# Autodesk Inventor assembly: ASY ДМФ лоток 050 илоотвод v2.0
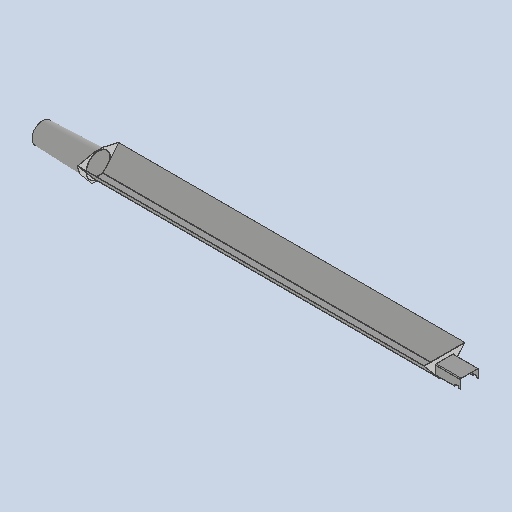
[picture p0: Inventor's stored thumbnail of the model, 512x512]
Saved by Autodesk Inventor 2026.2 (Build 302298000, 298)
## iProperties
Created: 2024-05-14
Part Number: ASY ДМФ лоток 050 илоотвод v2.0
Document SubType Name: Assembly
Designer: admin
Author: admin
## Documents named in this file (6)
- C:\Users\admin\Documents\Inventor\DMF-Disk-Micro-Filter\ASY ДМФ лоток 050 илоотвод v2.0.iam
- C:\Users\admin\Documents\Inventor\DMF-Disk-Micro-Filter\ДМФ 051 лоток илоотвод v2.0.ipt
- C:\Users\admin\Documents\Inventor\DMF-Disk-Micro-Filter\ДМФ 052 торец лотка кормовой v2.0.ipt
- C:\Users\admin\Documents\Inventor\DMF-Disk-Micro-Filter\ДМФ 053 швеллер лотка v2.0.ipt
- C:\Users\admin\Documents\Inventor\DMF-Disk-Micro-Filter\ДМФ 054 фланец лотка v2.0.ipt
- C:\Users\admin\Documents\Inventor\DMF-Disk-Micro-Filter\ДМФ 056 труба илоотвода v2.1.ipt
## Components (5 placed, 5 different names)
1. ДМФ 051 лоток илоотвод v2.0.ipt:1
2. ДМФ 052 торец лотка кормовой v2.0.ipt:1 — Flush:1, Mate:1
3. ДМФ 053 швеллер лотка v2.0.ipt:1 — Flush:1, Mate:1, Flush:2
4. ДМФ 056 труба илоотвода v2.1:1 — Rigid:4
5. ДМФ 054 фланец лотка v2.0.ipt:1 — Rigid:4
## Relationships (6: WeldJoint 3, Flush 2, Mate 1)
- [WeldJoint]: ДМФ 051 лоток илоотвод v2.0.ipt:1 ↔ ДМФ 052 торец лотка кормовой v2.0.ipt:1
- [WeldJoint]: ДМФ 051 лоток илоотвод v2.0.ipt:1 ↔ ДМФ 054 фланец лотка v2.0.ipt:1
- Flush:1 (20 mm): ДМФ 052 торец лотка кормовой v2.0.ipt:1 ↔ ДМФ 053 швеллер лотка v2.0.ipt:1
- Mate:1: ДМФ 052 торец лотка кормовой v2.0.ipt:1 ↔ ДМФ 053 швеллер лотка v2.0.ipt:1
- Flush:2: ДМФ 053 швеллер лотка v2.0.ipt:1
- Rigid:4 [WeldJoint]: ДМФ 056 труба илоотвода v2.1:1 ↔ ДМФ 054 фланец лотка v2.0.ipt:1
